# Autodesk Inventor assembly: PCBPT_V3
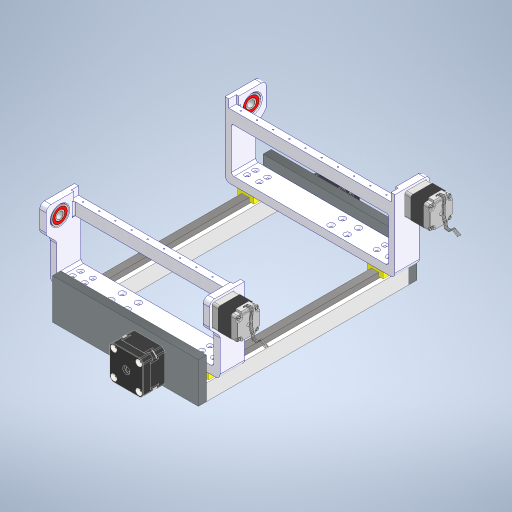
[picture p0: Inventor's stored thumbnail of the model, 512x512]
Saved by Autodesk Inventor 2024 (Build 280153000, 153)
## iProperties
Created: 2023-08-11
Part Number: PCBPT_V3
Document SubType Name: Assembly
Designer: l1534
Author: l1534
## Documents named in this file (10)
- C:\DATA\Documents\Lab\github\PCBPT\PCBPT_V3\Mechanical\PCBPT_V3.iam
- C:\DATA\Documents\Lab\github\PCBPT\PCBPT_V3\Mechanical\wall.ipt
- C:\DATA\Documents\Lab\github\PCBPT\PCBPT_V3\Mechanical\NEMA11\NEMA11.iam
- C:\DATA\Documents\Lab\github\PCBPT\PCBPT_V3\Mechanical\2020x260mm.ipt
- C:\DATA\Documents\Lab\github\PCBPT\PCBPT_V3\Mechanical\MGN9_rail.ipt
- C:\DATA\Documents\Lab\github\PCBPT\PCBPT_V3\Mechanical\MGN9C_block.ipt
- C:\DATA\Documents\Lab\github\PCBPT\PCBPT_V3\Mechanical\608-2RS Skate Board Ball Bearing\608-2RS Skate Board Ball Bearing.iam
- C:\DATA\Documents\Lab\github\PCBPT\PCBPT_V3\Mechanical\NEMA_17_PHB42S28-406A v2\NEMA_17_PHB42S28-406A v2.ipt
- C:\DATA\Documents\Lab\github\PCBPT\PCBPT_V3\Mechanical\gantry_R.ipt
- C:\DATA\Documents\Lab\github\PCBPT\PCBPT_V3\Mechanical\gantry_L_MIR.ipt
## Components (18 placed, 9 different names)
1. wall:1 — Rigid:1, Rigid:2, Flush:3, Mate:7
2. 2020x250mm:1 — Rigid:1, Rigid:5
3. 2020x250mm:2 — Rigid:2, Rigid:3, Rigid:4
4. wall:2 — Rigid:3, Flush:4, Mate:8
5. MGN9_rail:1 — Rigid:4, Slider:2, Slider:3
6. MGN9_rail:2 — Rigid:5, Slider:1, Slider:4
7. MGN9C_block:1 — Slider:4, Flush:2, Mate:12
8. MGN9C_block:2 — Slider:2, Flush:1, Mate:4
9. MGN9C_block:3 — Slider:1, Flush:1, Mate:5, Mate:6
10. MGN9C_block:4 — Slider:3, Flush:2, Mate:11, Mate:13
11. 608-2RS Skate Board Ball Bearing:2 [sub-assembly] — Mate:14, Mate:15
12. NEMA_17_PHB42S28-406A v2:1 — Flush:3, Mate:7
13. NEMA_17_PHB42S28-406A v2:2 — Flush:4, Mate:8
14. gantry_R:1 — Mate:4, Mate:5, Mate:6, Mate:9, Mate:10
15. NEMA11:5 [sub-assembly] — Mate:9
16. 608-2RS Skate Board Ball Bearing:3 [sub-assembly] — Mate:10
17. gantry_L_MIR:1 — Mate:11, Mate:12, Mate:13, Mate:14, Mate:15, Insert:1
18. NEMA11:6 [sub-assembly] — Insert:1
## Relationships (26: Mate 12, WeldJoint 5, TranslationJoint 4, Flush 4, Insert 1)
- Rigid:1 [WeldJoint]: wall:1 ↔ 2020x250mm:1
- Rigid:2 [WeldJoint]: wall:1 ↔ 2020x250mm:2
- Rigid:3 [WeldJoint]: 2020x250mm:2 ↔ wall:2
- Rigid:4 [WeldJoint]: 2020x250mm:2 ↔ MGN9_rail:1
- Rigid:5 [WeldJoint]: 2020x250mm:1 ↔ MGN9_rail:2
- Slider:1 [TranslationJoint]: MGN9_rail:2 ↔ MGN9C_block:3
- Slider:2 [TranslationJoint]: MGN9_rail:1 ↔ MGN9C_block:2
- Slider:3 [TranslationJoint]: MGN9_rail:1 ↔ MGN9C_block:4
- Slider:4 [TranslationJoint]: MGN9_rail:2 ↔ MGN9C_block:1
- Flush:1: MGN9C_block:2 ↔ MGN9C_block:3
- Flush:2: MGN9C_block:1 ↔ MGN9C_block:4
- Flush:3: wall:1 ↔ NEMA_17_PHB42S28-406A v2:1
- Flush:4: wall:2 ↔ NEMA_17_PHB42S28-406A v2:2
- Mate:4: MGN9C_block:2 ↔ gantry_R:1
- Mate:5: MGN9C_block:3 ↔ gantry_R:1
- Mate:6: MGN9C_block:3 ↔ gantry_R:1
- Mate:7: wall:1 ↔ NEMA_17_PHB42S28-406A v2:1
- Mate:8: wall:2 ↔ NEMA_17_PHB42S28-406A v2:2
- Mate:9: gantry_R:1 ↔ NEMA11:5
- Mate:10: gantry_R:1 ↔ 608-2RS Skate Board Ball Bearing:3
- Mate:11: MGN9C_block:4 ↔ gantry_L_MIR:1
- Mate:12: MGN9C_block:1 ↔ gantry_L_MIR:1
- Mate:13: MGN9C_block:4 ↔ gantry_L_MIR:1
- Mate:14: 608-2RS Skate Board Ball Bearing:2 ↔ gantry_L_MIR:1
- Mate:15: 608-2RS Skate Board Ball Bearing:2 ↔ gantry_L_MIR:1
- Insert:1: gantry_L_MIR:1 ↔ NEMA11:6
